# Autodesk Inventor assembly: RING_10
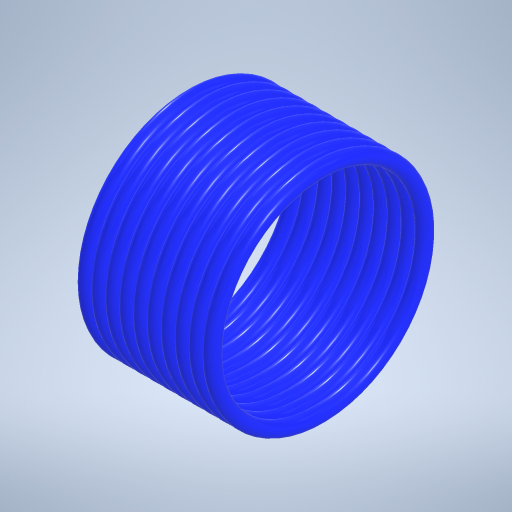
[picture p0: Inventor's stored thumbnail of the model, 512x512]
Saved by Autodesk Inventor 2023 (Build 270158000, 158)
## iProperties
Created: 2022-12-17
Part Number: RING_10
Document SubType Name: Assembly
Designer: blueh
Author: blueh
## Documents named in this file (2)
- C:\Users\blueh\OneDrive\デスクトップ\2023NHK_RR_1stvid\000_parts_zegi\NHK\RING_10.iam
- C:\Users\blueh\OneDrive\デスクトップ\2023NHK_RR_1stvid\3_car_saiki\ring_NHK23.ipt
## Components (10 placed, 1 different names)
1. ring_NHK23:1
2. ring_NHK23:2
3. ring_NHK23:3
4. ring_NHK23:4
5. ring_NHK23:5
6. ring_NHK23:6
7. ring_NHK23:7
8. ring_NHK23:8
9. ring_NHK23:9
10. ring_NHK23:10
## Component patterns: (10 elements, first: ring_NHK23:1)
